# Autodesk Inventor assembly: ship
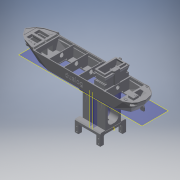
[picture p0: Inventor's stored thumbnail of the model, 180x180]
Saved by Autodesk Inventor 2018 (Build 220112000, 112)
## iProperties
Created: 2017-10-27
Part Number: ship
Document SubType Name: Assembly
Designer: erwin
Author: erwin
## Documents named in this file (4)
- D:\GitHub\SSJeVoisWheeledCargoShip\design\ship.iam
- D:\GitHub\SSJeVoisWheeledCargoShip\design\hull.ipt
- D:\GitHub\SSJeVoisWheeledCargoShip\design\holder.ipt
- D:\GitHub\SSJeVoisWheeledCargoShip\design\servo_bracket.ipt
## Components (3 placed, 3 different names)
1. hull:1 — Flush:1, Flush:2, Rigid:1
2. holder:1 — Flush:1, Flush:2, Flush:3, Rigid:1
3. servo_bracket:1 — Flush:3
## Relationships (4: Flush 3, WeldJoint 1)
- Flush:1: hull:1 ↔ holder:1
- Flush:2: hull:1 ↔ holder:1
- Flush:3: holder:1 ↔ servo_bracket:1
- Rigid:1 [WeldJoint]: hull:1 ↔ holder:1
